# Autodesk Inventor assembly: assembly
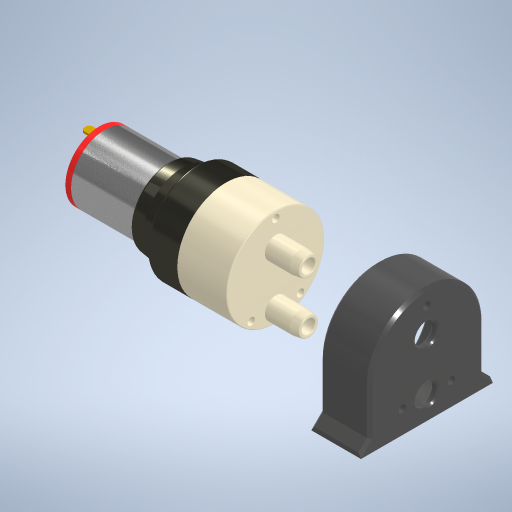
[picture p0: Inventor's stored thumbnail of the model, 512x512]
Saved by Autodesk Inventor 2024 (Build 280153000, 153)
## iProperties
Created: 2023-06-09
Part Number: assembly
Document SubType Name: Assembly
Designer: jeff7
Author: jeff7
## Documents named in this file (3)
- C:\Users\jeff7\Documents\GitHub\auto_garden\3D_printing\assembly.iam
- C:\Users\jeff7\Documents\GitHub\auto_garden\3D_printing\pump.ipt
- C:\Users\jeff7\Documents\GitHub\auto_garden\3D_printing\pump_socket_v2.ipt
## Components (2 placed, 2 different names)
1. pump:1 — Insert:1
2. pump_socket_v2:1 — Insert:1
## Relationships (1: Insert 1)
- Insert:1 (50.8 mm): pump:1 ↔ pump_socket_v2:1
